# Autodesk Inventor assembly: FINAL_MOP
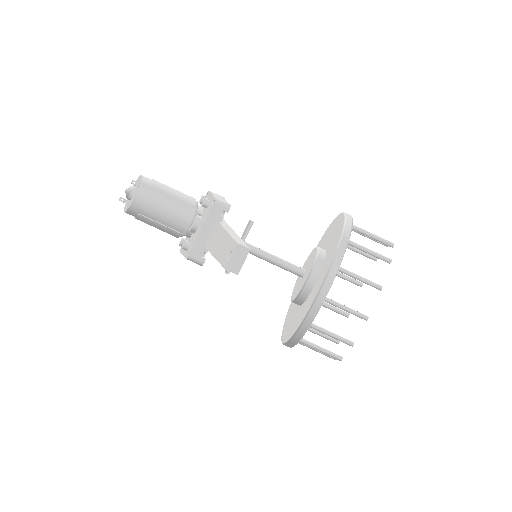
[picture p0: Inventor's stored thumbnail of the model, 512x512]
Saved by Autodesk Inventor 2022 (Build 260153000, 153)
## iProperties
Created: 2021-07-11
Part Number: FINAL_MOP
Document SubType Name: Assembly
Designer: Hp
Author: Hp
## Documents named in this file (5)
- C:\Users\LENOVO\Documents\Inventor\explo\FINAL_MOP.iam
- C:\Users\LENOVO\Documents\Inventor\explo\Orange MG555 12V 100RPM Square Gearbox DC motor.ipt
- C:\Users\LENOVO\Documents\Inventor\explo\horizontal_strip.ipt
- C:\Users\LENOVO\Documents\Inventor\explo\updated_base (2).ipt
- C:\Users\LENOVO\Documents\Inventor\explo\pin.ipt
## Components (4 placed, 4 different names)
1. Orange MG555 12V 100RPM Square Gearbox DC motor:1 — Rotational:1, Rotational:2, Rotational:3, Rotational:4, Rigid:1
2. horizontal_strip:1 — Rotational:1, Rotational:2, Rotational:3
3. updated_base (2):1 — Rotational:4
4. pin:1 — Rigid:1
## Relationships (5: RevoluteJoint 4, WeldJoint 1)
- Rotational:1 [RevoluteJoint]: Orange MG555 12V 100RPM Square Gearbox DC motor:1 ↔ horizontal_strip:1
- Rotational:2 [RevoluteJoint]: Orange MG555 12V 100RPM Square Gearbox DC motor:1 ↔ horizontal_strip:1
- Rotational:3 [RevoluteJoint]: Orange MG555 12V 100RPM Square Gearbox DC motor:1 ↔ horizontal_strip:1
- Rotational:4 [RevoluteJoint]: Orange MG555 12V 100RPM Square Gearbox DC motor:1 ↔ updated_base (2):1
- Rigid:1 [WeldJoint]: Orange MG555 12V 100RPM Square Gearbox DC motor:1 ↔ pin:1
